# Autodesk Inventor assembly: clino_build
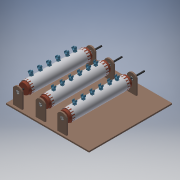
[picture p0: Inventor's stored thumbnail of the model, 180x180]
Saved by Autodesk Inventor 2018 (Build 220112000, 112)
## iProperties
Created: 2018-09-09
Part Number: clino_build
Document SubType Name: Assembly
Designer: Fredy Espana C
Author: Fredy Espana C
## Documents named in this file (8)
- C:\Users\Fredy Espana C\Documents\Inventor\Clino\clino_build.iam
- C:\Users\Fredy Espana C\Documents\Inventor\Clino\2inpvc_pipe.ipt
- C:\Users\Fredy Espana C\Documents\Inventor\Clino\pipe_holder.ipt
- C:\Users\Fredy Espana C\Documents\Inventor\Clino\snap_grip.ipt
- C:\Users\Fredy Espana C\Documents\Inventor\Clino\mdf_support.ipt
- C:\Users\Fredy Espana C\Documents\Inventor\Clino\shaft.ipt
- C:\Users\Fredy Espana C\Documents\Inventor\Clino\lib\en-US\Bearing GB_T 292-2007\Rolling bearing B706 C GB_T 292-2007.ipt
- C:\Users\Fredy Espana C\Documents\Inventor\Clino\base_plank.ipt
## Components (43 placed, 7 different names)
1. 2inpvc_pipe:1 — Mate:1, Mate:2, Cylindrical:1, Cylindrical:2, Insert:1, Insert:2, Insert:3, Insert:4, Insert:5, Insert:6
2. pipe_holder:1 — Mate:1, Cylindrical:2, Cylindrical:3
3. pipe_holder:2 — Mate:2, Cylindrical:1
4. snap_grip:1 — Insert:1
5. snap_grip:2 — Insert:2
6. snap_grip:3 — Insert:3
7. snap_grip:4 — Insert:4
8. snap_grip:5 — Insert:5
9. snap_grip:6 — Insert:6
10. shaft:1 — Cylindrical:3, Mate:4, Cylindrical:4
11. mdf_support:1 — Mate:3, Flush:1, Flush:2, Flush:3, Mate:16
12. mdf_support:2 — Flush:2, Flush:3, Mate:5, Flush:4
13. Bearing GB/T 292-2007 Type IN - withdrawn B706 C:3 — Mate:3, Mate:4, Flush:1, Cylindrical:4
14. Bearing GB/T 292-2007 Type IN - withdrawn B706 C:4 — Mate:5, Flush:4
15. 2inpvc_pipe:2
16. pipe_holder:3
17. pipe_holder:4
18. snap_grip:7
19. snap_grip:8
20. snap_grip:9
21. snap_grip:10
22. snap_grip:11
23. snap_grip:12
24. shaft:2
25. mdf_support:3 — Mate:18
26. mdf_support:4
27. Bearing GB/T 292-2007 Type IN - withdrawn B706 C:5
28. Bearing GB/T 292-2007 Type IN - withdrawn B706 C:6
29. 2inpvc_pipe:3
30. pipe_holder:5
31. pipe_holder:6
32. snap_grip:13
33. snap_grip:14
34. snap_grip:15
35. snap_grip:16
36. snap_grip:17
37. snap_grip:18
38. shaft:3
39. mdf_support:5 — Mate:17
40. mdf_support:6
41. Bearing GB/T 292-2007 Type IN - withdrawn B706 C:7
42. Bearing GB/T 292-2007 Type IN - withdrawn B706 C:8
43. base_plank:1 — Mate:16, Mate:17, Mate:18
## Relationships (60: Mate 18, Insert 18, CylindricalJoint 12, Flush 12)
- Mate:1: 2inpvc_pipe:1 ↔ pipe_holder:1
- Mate:2: 2inpvc_pipe:1 ↔ pipe_holder:2
- Cylindrical:1: 2inpvc_pipe:1 ↔ pipe_holder:2
- Cylindrical:2: 2inpvc_pipe:1 ↔ pipe_holder:1
- Insert:1 (-38.1 mm): 2inpvc_pipe:1 ↔ snap_grip:1
- Insert:2 (-76.2 mm): 2inpvc_pipe:1 ↔ snap_grip:2
- Insert:3 (-114.3 mm): 2inpvc_pipe:1 ↔ snap_grip:3
- Insert:4 (-107.95 mm): 2inpvc_pipe:1 ↔ snap_grip:4
- Insert:5 (-69.85 mm): 2inpvc_pipe:1 ↔ snap_grip:5
- Insert:6 (-38.1 mm): 2inpvc_pipe:1 ↔ snap_grip:6
- Cylindrical:3: pipe_holder:1 ↔ shaft:1
- Mate:3: mdf_support:1 ↔ Bearing GB/T 292-2007 Type IN - withdrawn B706 C:3
- Mate:4: shaft:1 ↔ Bearing GB/T 292-2007 Type IN - withdrawn B706 C:3
- Flush:1: mdf_support:1 ↔ Bearing GB/T 292-2007 Type IN - withdrawn B706 C:3
- Cylindrical:4: shaft:1 ↔ Bearing GB/T 292-2007 Type IN - withdrawn B706 C:3
- Flush:2: mdf_support:1 ↔ mdf_support:2
- Flush:3: mdf_support:1 ↔ mdf_support:2
- Mate:5: mdf_support:2 ↔ Bearing GB/T 292-2007 Type IN - withdrawn B706 C:4
- Flush:4: mdf_support:2 ↔ Bearing GB/T 292-2007 Type IN - withdrawn B706 C:4
- [Mate]: 2inpvc_pipe:2 ↔ pipe_holder:3
- [Mate]: 2inpvc_pipe:2 ↔ pipe_holder:4
- [CylindricalJoint]: 2inpvc_pipe:2 ↔ pipe_holder:4
- [CylindricalJoint]: 2inpvc_pipe:2 ↔ pipe_holder:3
- [Insert] (-38.1 mm): 2inpvc_pipe:2 ↔ snap_grip:7
- [Insert] (-76.2 mm): 2inpvc_pipe:2 ↔ snap_grip:8
- [Insert] (-114.3 mm): 2inpvc_pipe:2 ↔ snap_grip:9
- [Insert] (-107.95 mm): 2inpvc_pipe:2 ↔ snap_grip:10
- [Insert] (-69.85 mm): 2inpvc_pipe:2 ↔ snap_grip:11
- [Insert] (-38.1 mm): 2inpvc_pipe:2 ↔ snap_grip:12
- [CylindricalJoint]: pipe_holder:3 ↔ shaft:2
- [Mate]: mdf_support:3 ↔ Bearing GB/T 292-2007 Type IN - withdrawn B706 C:5
- [Mate]: shaft:2 ↔ Bearing GB/T 292-2007 Type IN - withdrawn B706 C:5
- [Flush]: mdf_support:3 ↔ Bearing GB/T 292-2007 Type IN - withdrawn B706 C:5
- [CylindricalJoint]: shaft:2 ↔ Bearing GB/T 292-2007 Type IN - withdrawn B706 C:5
- [Flush]: mdf_support:3 ↔ mdf_support:4
- [Flush]: mdf_support:3 ↔ mdf_support:4
- [Mate]: mdf_support:4 ↔ Bearing GB/T 292-2007 Type IN - withdrawn B706 C:6
- [Flush]: mdf_support:4 ↔ Bearing GB/T 292-2007 Type IN - withdrawn B706 C:6
- [Mate]: 2inpvc_pipe:3 ↔ pipe_holder:5
- [Mate]: 2inpvc_pipe:3 ↔ pipe_holder:6
- [CylindricalJoint]: 2inpvc_pipe:3 ↔ pipe_holder:6
- [CylindricalJoint]: 2inpvc_pipe:3 ↔ pipe_holder:5
- [Insert] (-38.1 mm): 2inpvc_pipe:3 ↔ snap_grip:13
- [Insert] (-76.2 mm): 2inpvc_pipe:3 ↔ snap_grip:14
- [Insert] (-114.3 mm): 2inpvc_pipe:3 ↔ snap_grip:15
- [Insert] (-107.95 mm): 2inpvc_pipe:3 ↔ snap_grip:16
- [Insert] (-69.85 mm): 2inpvc_pipe:3 ↔ snap_grip:17
- [Insert] (-38.1 mm): 2inpvc_pipe:3 ↔ snap_grip:18
- [CylindricalJoint]: pipe_holder:5 ↔ shaft:3
- [Mate]: mdf_support:5 ↔ Bearing GB/T 292-2007 Type IN - withdrawn B706 C:7
- [Mate]: shaft:3 ↔ Bearing GB/T 292-2007 Type IN - withdrawn B706 C:7
- [Flush]: mdf_support:5 ↔ Bearing GB/T 292-2007 Type IN - withdrawn B706 C:7
- [CylindricalJoint]: shaft:3 ↔ Bearing GB/T 292-2007 Type IN - withdrawn B706 C:7
- [Flush]: mdf_support:5 ↔ mdf_support:6
- [Flush]: mdf_support:5 ↔ mdf_support:6
- [Mate]: mdf_support:6 ↔ Bearing GB/T 292-2007 Type IN - withdrawn B706 C:8
- [Flush]: mdf_support:6 ↔ Bearing GB/T 292-2007 Type IN - withdrawn B706 C:8
- Mate:16: mdf_support:1 ↔ base_plank:1
- Mate:17: mdf_support:5 ↔ base_plank:1
- Mate:18: mdf_support:3 ↔ base_plank:1
## Named parameters: d31_d21 = 0 mm, d32_d22 = -44.534332 deg, d33_d23 = -0.3 mm, d34_d24 = 0 mm, d35_d25 = 0 mm, d36_d28 = 0 mm, d37_d30 = 0 mm, d38_d5 = 6 mm, d39_d6 = -38.1 mm, d40_d7 = -76.2 mm, d41_d8 = -114.3 mm, d42_d9 = -107.95 mm, d43_d10 = -69.85 mm, d44_d11 = -38.1 mm, d45_d14 = 80.869627 deg, d46_d15 = -5.03126 mm, d47_d19 = 0 mm, d48_d20 = 0 mm, d49_d0 = 0 mm, d50_d1 = 0 mm, d51_d2 = -64.512651 deg, d52_d3 = -12 mm, d53_d4 = -64.517879 deg, d54_d21 = 0 mm, d55_d22 = -44.348314 deg, d56_d23 = -0.3 mm, d57_d24 = 0 mm, d58_d25 = 0 mm, d59_d28 = 0 mm, d60_d30 = 0 mm, d61_d5 = 6 mm, d62_d6 = -38.1 mm, d63_d7 = -76.2 mm, d64_d8 = -114.3 mm, d65_d9 = -107.95 mm, d66_d10 = -69.85 mm, d67_d11 = -38.1 mm, d68_d14 = 80.683609 deg, d69_d15 = -8.58752 mm, d70_d19 = 0 mm, d71_d20 = 0 mm, d72_d0 = 0 mm, d73_d1 = 0 mm, d74_d2 = -42.114766 deg, d75_d3 = -12 mm, d76_d4 = -42.114766 deg
